# Autodesk Inventor assembly: ARM
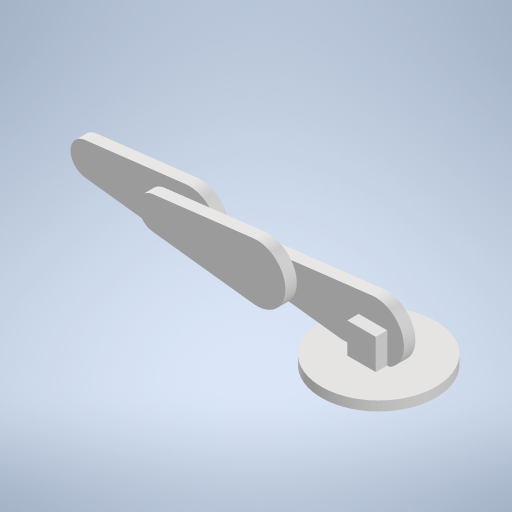
[picture p0: Inventor's stored thumbnail of the model, 512x512]
Saved by Autodesk Inventor 2023.2 (Build 272271000, 271)
## iProperties
Created: 2022-12-11
Part Number: ARM
Document SubType Name: Assembly
Designer: Team 4026
Author: Team 4026
## Documents named in this file (3)
- C:\Users\Team 4026\Documents\ARM.iam
- C:\Users\Team 4026\Documents\Arm holder.ipt
- C:\Users\Team 4026\Documents\Arm.ipt
## Components (4 placed, 2 different names)
1. Arm holder:1 — Mate:1
2. Arm:1 — Mate:1, Mate:2
3. Arm:2 — Mate:2, Mate:3
4. Arm:3 — Mate:3
## Relationships (3: Mate 3)
- Mate:1: Arm holder:1 ↔ Arm:1
- Mate:2: Arm:1 ↔ Arm:2
- Mate:3: Arm:2 ↔ Arm:3
